# Autodesk Inventor assembly: MontagemPlug
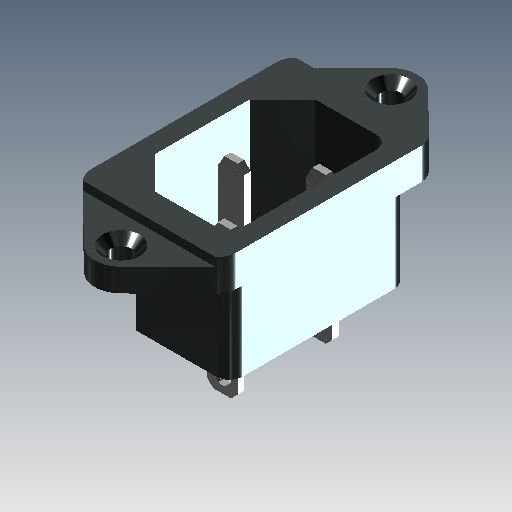
[picture p0: Inventor's stored thumbnail of the model, 512x512]
Saved by Autodesk Inventor 2020 (Build 240168000, 168)
## iProperties
Created: 2015-09-19
Part Number: MontagemPlug
Document SubType Name: Assembly
Designer: Elvis Mayk
Author: Elvis Mayk
## Documents named in this file (4)
- C:\Users\Hernan\Documents\Router CNC\Diseños Autodesk Inventor\Ensambles\RouterCNC 8-7-20\8-7-2020-V2\Ensamble fino 2\Botonera\Botonera 2\Botonera\Interlock\MontagemPlug.iam
- C:\Users\Hernan\Documents\Router CNC\Diseños Autodesk Inventor\Ensambles\RouterCNC 8-7-20\8-7-2020-V2\Ensamble fino 2\Botonera\Botonera 2\Botonera\Interlock\PlacaFasePlug.ipt
- C:\Users\Hernan\Documents\Router CNC\Diseños Autodesk Inventor\Ensambles\RouterCNC 8-7-20\8-7-2020-V2\Ensamble fino 2\Botonera\Botonera 2\Botonera\Interlock\PlugFemeaTomada.ipt
- C:\Users\Hernan\Documents\Router CNC\Diseños Autodesk Inventor\Ensambles\RouterCNC 8-7-20\8-7-2020-V2\Ensamble fino 2\Botonera\Botonera 2\Botonera\Interlock\PlacaTerraPlug.ipt
## Components (4 placed, 3 different names)
1. PlugFemeaTomada:1 — Mate:1, Mate:2, Mate:3, Mate:4, Mate:5, Mate:6
2. PlacaFasePlug:1 — Flush:1, Flush:2, Mate:1, Mate:2, Flush:3
3. PlacaFasePlug:2 — Flush:1, Flush:3, Mate:3, Mate:4
4. PlacaTerraPlug:1 — Flush:2, Mate:5, Mate:6
## Relationships (9: Mate 6, Flush 3)
- Flush:1: PlacaFasePlug:1 ↔ PlacaFasePlug:2
- Flush:2: PlacaFasePlug:1 ↔ PlacaTerraPlug:1
- Mate:1: PlugFemeaTomada:1 ↔ PlacaFasePlug:1
- Mate:2: PlugFemeaTomada:1 ↔ PlacaFasePlug:1
- Flush:3: PlacaFasePlug:1 ↔ PlacaFasePlug:2
- Mate:3: PlugFemeaTomada:1 ↔ PlacaFasePlug:2
- Mate:4: PlugFemeaTomada:1 ↔ PlacaFasePlug:2
- Mate:5: PlugFemeaTomada:1 ↔ PlacaTerraPlug:1
- Mate:6: PlugFemeaTomada:1 ↔ PlacaTerraPlug:1
